# Autodesk Inventor assembly: Assembly1
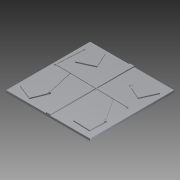
[picture p0: Inventor's stored thumbnail of the model, 180x180]
Saved by Autodesk Inventor 2011 (Build 150239000, 239)
## iProperties
Created: 2011-07-10
Part Number: Assembly1
Document SubType Name: Assembly
Designer: adowning
Author: adowning
## Documents named in this file (5)
- C:\Documents and Settings\adowning.ST-USERS\My Documents\private\matthew\prlite\base\wheelrot test\Assembly1.iam
- C:\Documents and Settings\adowning.ST-USERS\My Documents\private\matthew\prlite\base\wheelrot test\base.ipt
- C:\Documents and Settings\adowning.ST-USERS\My Documents\private\matthew\prlite\base\wheelrot test\lasiness.ipt
- C:\Documents and Settings\adowning.ST-USERS\My Documents\private\matthew\prlite\base\wheelrot test\bar2.ipt
- C:\Documents and Settings\adowning.ST-USERS\My Documents\private\matthew\prlite\base\wheelrot test\connection.ipt
## Components (10 placed, 4 different names)
1. base:1 — Mate:1, Mate:2, Mate:3, Mate:4, Mate:5, Mate:6, Flush:1, Mate:7
2. lasiness:1 — Mate:4, Mate:5, Mate:11, Mate:12
3. lasiness:2 — Mate:3, Mate:6, Mate:10, Mate:15
4. lasiness:3 — Mate:2, Mate:7, Mate:8, Mate:13
5. lasiness:4 — Mate:1, Flush:1, Mate:9, Mate:14
6. bar2:1 — Mate:8, Mate:13, Mate:17
7. bar2:2 — Mate:11, Mate:12, Mate:18, Mate:20
8. bar2:3 — Mate:10, Mate:15, Mate:19
9. bar2:4 — Mate:9, Mate:14, Mate:16
10. connection:1 — Mate:16, Mate:17, Mate:18, Mate:19, Mate:20
## Relationships (21: Mate 20, Flush 1)
- Mate:1: base:1 ↔ lasiness:4
- Mate:2: base:1 ↔ lasiness:3
- Mate:3: base:1 ↔ lasiness:2
- Mate:4: base:1 ↔ lasiness:1
- Mate:5: base:1 ↔ lasiness:1
- Mate:6: base:1 ↔ lasiness:2
- Flush:1: base:1 ↔ lasiness:4
- Mate:7: base:1 ↔ lasiness:3
- Mate:8: lasiness:3 ↔ bar2:1
- Mate:9: lasiness:4 ↔ bar2:4
- Mate:10: lasiness:2 ↔ bar2:3
- Mate:11: lasiness:1 ↔ bar2:2
- Mate:12: lasiness:1 ↔ bar2:2
- Mate:13: lasiness:3 ↔ bar2:1
- Mate:14: lasiness:4 ↔ bar2:4
- Mate:15: lasiness:2 ↔ bar2:3
- Mate:16: bar2:4 ↔ connection:1
- Mate:17: bar2:1 ↔ connection:1
- Mate:18: bar2:2 ↔ connection:1
- Mate:19: bar2:3 ↔ connection:1
- Mate:20: bar2:2 ↔ connection:1
